# Autodesk Inventor assembly: Configuration 1
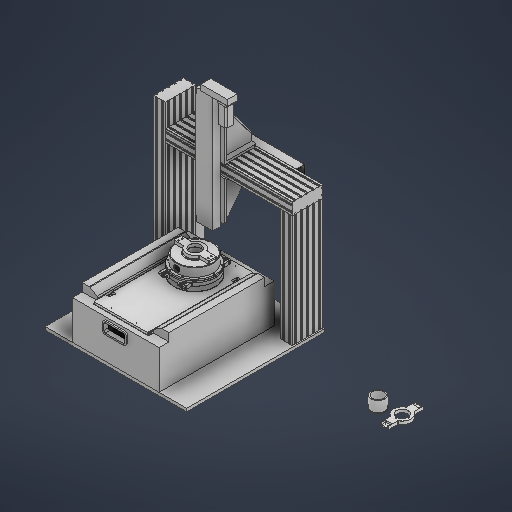
[picture p0: Inventor's stored thumbnail of the model, 512x512]
Saved by Autodesk Inventor 2025 (Build 290162000, 162)
## iProperties
Created: 2024-06-05
Part Number: Configuration 1
Document SubType Name: Assembly
Designer: AdminForWorker
Title: Printer Assembly v13
Author: AdminForWorker
## Documents named in this file (18)
- C:\Users\mayhe\OneDrive\Documents\GitHub\In-situ-monitoring-of-powder-bed-fusion-additive-manufacturing\system_development\Orichalcum\v0.2\Hardware_design\Full Printer Assembly\Printer Assembly.iam
- C:\Users\mayhe\OneDrive\Documents\GitHub\In-situ-monitoring-of-powder-bed-fusion-additive-manufacturing\system_development\Orichalcum\v0.2\Hardware_design\Full Printer Assembly\Printer Body v6.ipt
- C:\Users\mayhe\OneDrive\Documents\GitHub\In-situ-monitoring-of-powder-bed-fusion-additive-manufacturing\system_development\Orichalcum\v0.2\Hardware_design\Full Printer Assembly\Printer Frame.ipt
- C:\Users\mayhe\OneDrive\Documents\GitHub\In-situ-monitoring-of-powder-bed-fusion-additive-manufacturing\system_development\Orichalcum\v0.2\Hardware_design\Full Printer Assembly\overhead laser unit v1.ipt
- C:\Users\mayhe\OneDrive\Documents\GitHub\In-situ-monitoring-of-powder-bed-fusion-additive-manufacturing\system_development\Orichalcum\v0.2\Hardware_design\Full Printer Assembly\Part4.ipt
- C:\Users\mayhe\OneDrive\Documents\GitHub\In-situ-monitoring-of-powder-bed-fusion-additive-manufacturing\system_development\Orichalcum\v0.2\Hardware_design\custom-cover\cover\Updated Cover.ipt
- C:\Users\mayhe\OneDrive\Documents\GitHub\In-situ-monitoring-of-powder-bed-fusion-additive-manufacturing\system_development\Orichalcum\v0.2\Hardware_design\custom-cover\cylinder-parts\final-parts\Cylinder Bottom Ring.ipt
- C:\Users\mayhe\OneDrive\Documents\GitHub\In-situ-monitoring-of-powder-bed-fusion-additive-manufacturing\system_development\Orichalcum\v0.2\Hardware_design\custom-cover\cylinder-parts\final-parts\Cylinder Slidey Bit Housing.ipt
- C:\Users\mayhe\OneDrive\Documents\GitHub\In-situ-monitoring-of-powder-bed-fusion-additive-manufacturing\system_development\Orichalcum\v0.2\Hardware_design\custom-cover\cylinder-parts\Cylinder 80-20 Spacer_1.ipt
- C:\Users\mayhe\OneDrive\Documents\GitHub\In-situ-monitoring-of-powder-bed-fusion-additive-manufacturing\system_development\Orichalcum\v0.2\Hardware_design\custom-cover\cylinder-parts\Cylinder 80-20 Spacer_2.ipt
- C:\Users\mayhe\OneDrive\Documents\GitHub\In-situ-monitoring-of-powder-bed-fusion-additive-manufacturing\system_development\Orichalcum\v0.2\Hardware_design\custom-cover\8020-parts\20-2020-300.ipt
- C:\Users\mayhe\OneDrive\Documents\GitHub\In-situ-monitoring-of-powder-bed-fusion-additive-manufacturing\system_development\Orichalcum\v0.2\Hardware_design\custom-cover\cylinder-parts\cylinder-segments\Cylinder Segment .ipt
- C:\Users\mayhe\OneDrive\Documents\GitHub\In-situ-monitoring-of-powder-bed-fusion-additive-manufacturing\system_development\Orichalcum\v0.2\Hardware_design\custom-cover\cylinder-parts\final-parts\Cylinder Segment - 01.ipt
- C:\Users\mayhe\OneDrive\Documents\GitHub\In-situ-monitoring-of-powder-bed-fusion-additive-manufacturing\system_development\Orichalcum\v0.2\Hardware_design\custom-cover\cylinder-parts\final-parts\Cylinder Segment - Face.ipt
- C:\Users\mayhe\OneDrive\Documents\GitHub\In-situ-monitoring-of-powder-bed-fusion-additive-manufacturing\system_development\Orichalcum\v0.2\Hardware_design\custom-cover\cylinder-parts\final-parts\Cylinder Segment - 09.ipt
- C:\Users\mayhe\OneDrive\Documents\GitHub\In-situ-monitoring-of-powder-bed-fusion-additive-manufacturing\system_development\Orichalcum\v0.2\Hardware_design\custom-cover\cylinder-parts\final-parts\Cylinder Segment - 10.ipt
- C:\Users\mayhe\OneDrive\Documents\GitHub\In-situ-monitoring-of-powder-bed-fusion-additive-manufacturing\system_development\Orichalcum\v0.2\Hardware_design\custom-cover\cylinder-parts\cylinder-segments\Head Thing.ipt
- C:\Users\mayhe\OneDrive\Documents\GitHub\In-situ-monitoring-of-powder-bed-fusion-additive-manufacturing\system_development\Orichalcum\v0.2\Hardware_design\custom-cover\cylinder-parts\cylinder-segments\Cylinder Segment - Face.ipt
## Components (20 placed, 15 different names)
1. Printer Frame:1 — Flush:1, Mate:1, Mate:2, Mate:3, Flush:2, Flush:3
2. Printer Body v6:1 — Flush:1, Mate:1, Mate:2, Mate:5, Mate:6, Mate:7
3. overhead laser unit v1:1 — Mate:4, Angle:1, Flush:4
4. Part4:1 — Mate:3, Flush:2, Flush:3, Mate:4, Angle:1, Flush:4
5. Updated Cover:1 — Mate:5, Mate:6, Mate:7, Rotational:4, Mate:53
6. Cylinder 80-20 Spacer_1:2 — Flush:5, Mate:29, Flush:6, Mate:30, Mate:59
7. Cylinder 80-20 Spacer_2:1 — Mate:26, Mate:60, Mate:61, Mate:62
8. Cylinder 80-20 Spacer_2:2 — Mate:47, Mate:54, Mate:55, Mate:56, Flush:7, Mate:57
9. Cylinder 80-20 Spacer_1:3 — Mate:64, Mate:65, Mate:66
10. 20-2020-300:1 — Mate:29, Flush:6, Mate:56, Flush:7, Mate:58
11. 20-2020-300:2 — Mate:26, Flush:5, Mate:52, Mate:63
12. Cylinder Segment - 01:1 — Mate:30, Mate:47, Rotational:2, Mate:48
13. Cylinder Slidey Bit Housing:1 — Rotational:2, Mate:48, Mate:49, Mate:50, Mate:51
14. Cylinder Segment - Face:2 — Mate:49, Rotational:3
15. Cylinder Segment - 09:3 — Mate:51, Mate:52
16. Cylinder Segment - 10:4 — Mate:50
17. Head Thing:1 — Rotational:3
18. Cylinder Bottom Ring:1 — Rotational:4, Mate:53, Mate:54, Mate:55, Mate:57, Mate:58, Mate:59, Mate:60, Mate:61, Mate:62, Mate:63, Mate:64, Mate:65, Mate:66
19. Cylinder Segment - Face:5
20. Head Thing:2
## Relationships (41: Mate 30, Flush 7, RevoluteJoint 3, Angle 1)
- Flush:1: Printer Frame:1 ↔ Printer Body v6:1
- Mate:1: Printer Frame:1 ↔ Printer Body v6:1
- Mate:2 (92.5 mm): Printer Frame:1 ↔ Printer Body v6:1
- Mate:3: Printer Frame:1 ↔ Part4:1
- Flush:2 (28.5 mm): Printer Frame:1 ↔ Part4:1
- Flush:3 (-27 mm): Printer Frame:1 ↔ Part4:1
- Mate:4: overhead laser unit v1:1 ↔ Part4:1
- Angle:1 (179.9998 deg): overhead laser unit v1:1 ↔ Part4:1
- Flush:4 (-30 mm): overhead laser unit v1:1 ↔ Part4:1
- Mate:5: Printer Body v6:1 ↔ Updated Cover:1
- Mate:6: Printer Body v6:1 ↔ Updated Cover:1
- Mate:7: Printer Body v6:1 ↔ Updated Cover:1
- Mate:26: Cylinder 80-20 Spacer_2:1 ↔ 20-2020-300:2
- Flush:5: Cylinder 80-20 Spacer_1:2 ↔ 20-2020-300:2
- Mate:29: Cylinder 80-20 Spacer_1:2 ↔ 20-2020-300:1
- Flush:6: Cylinder 80-20 Spacer_1:2 ↔ 20-2020-300:1
- Mate:30: Cylinder 80-20 Spacer_1:2 ↔ Cylinder Segment - 01:1
- Mate:47: Cylinder 80-20 Spacer_2:2 ↔ Cylinder Segment - 01:1
- Rotational:2 [RevoluteJoint]: Cylinder Segment - 01:1 ↔ Cylinder Slidey Bit Housing:1
- Mate:48: Cylinder Segment - 01:1 ↔ Cylinder Slidey Bit Housing:1
- Mate:49: Cylinder Slidey Bit Housing:1 ↔ Cylinder Segment - Face:2
- Mate:50: Cylinder Slidey Bit Housing:1 ↔ Cylinder Segment - 10:4
- Mate:51: Cylinder Slidey Bit Housing:1 ↔ Cylinder Segment - 09:3
- Mate:52: 20-2020-300:2 ↔ Cylinder Segment - 09:3
- Rotational:3 [RevoluteJoint]: Cylinder Segment - Face:2 ↔ Head Thing:1
- Rotational:4 [RevoluteJoint]: Updated Cover:1 ↔ Cylinder Bottom Ring:1
- Mate:53: Updated Cover:1 ↔ Cylinder Bottom Ring:1
- Mate:54: Cylinder 80-20 Spacer_2:2 ↔ Cylinder Bottom Ring:1
- Mate:55: Cylinder 80-20 Spacer_2:2 ↔ Cylinder Bottom Ring:1
- Mate:56: Cylinder 80-20 Spacer_2:2 ↔ 20-2020-300:1
- Flush:7: Cylinder 80-20 Spacer_2:2 ↔ 20-2020-300:1
- Mate:57: Cylinder 80-20 Spacer_2:2 ↔ Cylinder Bottom Ring:1
- Mate:58: 20-2020-300:1 ↔ Cylinder Bottom Ring:1
- Mate:59: Cylinder 80-20 Spacer_1:2 ↔ Cylinder Bottom Ring:1
- Mate:60: Cylinder 80-20 Spacer_2:1 ↔ Cylinder Bottom Ring:1
- Mate:61: Cylinder 80-20 Spacer_2:1 ↔ Cylinder Bottom Ring:1
- Mate:62: Cylinder 80-20 Spacer_2:1 ↔ Cylinder Bottom Ring:1
- Mate:63: 20-2020-300:2 ↔ Cylinder Bottom Ring:1
- Mate:64: Cylinder 80-20 Spacer_1:3 ↔ Cylinder Bottom Ring:1
- Mate:65: Cylinder 80-20 Spacer_1:3 ↔ Cylinder Bottom Ring:1
- Mate:66: Cylinder 80-20 Spacer_1:3 ↔ Cylinder Bottom Ring:1
